# Autodesk Inventor assembly: IMX291 Camera Case Assembly
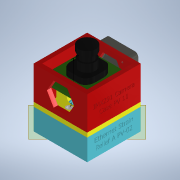
[picture p0: Inventor's stored thumbnail of the model, 180x180]
Saved by Autodesk Inventor 2022.1 (Build 261234000, 234)
## iProperties
Created: 2021-07-23
Part Number: IMX291 Camera Case Assembly
Document SubType Name: Assembly
Designer: robst
Author: robst
## Documents named in this file (10)
- C:\git\CAD-Development\robSteele\ShapeWays\GlobalMeteorNetwork\IMX291 Camera Case Assembly.iam
- C:\git\CAD-Development\robSteele\ShapeWays\GlobalMeteorNetwork\IMX291 Camera Case Base.ipt
- C:\git\CAD-Development\robSteele\ShapeWays\GlobalMeteorNetwork\IMX291 Camera.ipt
- C:\Users\robst\Documents\Inventor\Content Center Files\R2021\en-US\U UNC 2605\Unbrako - 2 x 1_2 - 56(10).ipt
- C:\git\CAD-Development\robSteele\ShapeWays\GlobalMeteorNetwork\IMX291 Camera Case Bottom.ipt
- C:\git\CAD-Development\robSteele\ShapeWays\GlobalMeteorNetwork\IMX291 Ethernet Cable Strain Relief.ipt
- c:\git\CAD-MfgResources\McMaster-Carr\Insert\6-32x0.281_94459A290_NO THREADS_Brass Heat-Set Inserts for Plastic.ipt
- c:\git\CAD-MfgResources\McMaster-Carr\Button Screw\6-32\6-32 x 1_000 92949A153_18-8 Stainless Steel Button Head Hex Drive Screw.ipt
- c:\git\CAD-MfgResources\McMaster-Carr\Washer\Number_6_Washer\90107A007_TYPE 316 STAINLESS STEEL FLAT WASHER.ipt
- C:\git\CAD-Development\robSteele\ShapeWays\GlobalMeteorNetwork\LD3007MS FAN.ipt
## Components (12 placed, 9 different names)
1. IMX291 Camera Case Base:1 — Insert:1, Insert:2, Mate:3, Flush:1, Flush:2, Insert:9, Insert:10
2. IMX291 Camera:1 — Insert:1, Insert:2, Mate:1, Mate:2
3. Unbrako UNC Hex Socket Button Cap - Inch 2 x 1/2:1 — Mate:1, Mate:2
4. IMX291 Camera Case Bottom:1 — Mate:3, Flush:1, Flush:2, Mate:4, Flush:3, Flush:4, Insert:3, Insert:4, Insert:5, Insert:6
5. IMX291 Ethernet Cable Strain Relief:1 — Mate:4, Flush:3, Flush:4, Insert:7
6. 6-32x0.281_94459A290_NO THREADS_Brass Heat-Set Inserts for Plastic:1 — Insert:3
7. 6-32x0.281_94459A290_NO THREADS_Brass Heat-Set Inserts for Plastic:2 — Insert:4
8. 6-32x0.281_94459A290_NO THREADS_Brass Heat-Set Inserts for Plastic:3 — Insert:5
9. 6-32x0.281_94459A290_NO THREADS_Brass Heat-Set Inserts for Plastic:4 — Insert:6
10. 6-32 x 1_000 92949A153_18-8 Stainless Steel Button Head Hex Drive Screw:1 — Insert:8
11. 90107A007_TYPE 316 STAINLESS STEEL FLAT WASHER:1 — Insert:7, Insert:8
12. LD3007MS FAN:1 — Insert:9, Insert:10
## Relationships (18: Insert 10, Mate 4, Flush 4)
- Insert:1: IMX291 Camera Case Base:1 ↔ IMX291 Camera:1
- Insert:2: IMX291 Camera Case Base:1 ↔ IMX291 Camera:1
- Mate:1: IMX291 Camera:1 ↔ Unbrako UNC Hex Socket Button Cap - Inch 2 x 1/2:1
- Mate:2: IMX291 Camera:1 ↔ Unbrako UNC Hex Socket Button Cap - Inch 2 x 1/2:1
- Mate:3: IMX291 Camera Case Base:1 ↔ IMX291 Camera Case Bottom:1
- Flush:1: IMX291 Camera Case Base:1 ↔ IMX291 Camera Case Bottom:1
- Flush:2: IMX291 Camera Case Base:1 ↔ IMX291 Camera Case Bottom:1
- Mate:4: IMX291 Camera Case Bottom:1 ↔ IMX291 Ethernet Cable Strain Relief:1
- Flush:3: IMX291 Camera Case Bottom:1 ↔ IMX291 Ethernet Cable Strain Relief:1
- Flush:4: IMX291 Camera Case Bottom:1 ↔ IMX291 Ethernet Cable Strain Relief:1
- Insert:3: IMX291 Camera Case Bottom:1 ↔ 6-32x0.281_94459A290_NO THREADS_Brass Heat-Set Inserts for Plastic:1
- Insert:4: IMX291 Camera Case Bottom:1 ↔ 6-32x0.281_94459A290_NO THREADS_Brass Heat-Set Inserts for Plastic:2
- Insert:5: IMX291 Camera Case Bottom:1 ↔ 6-32x0.281_94459A290_NO THREADS_Brass Heat-Set Inserts for Plastic:3
- Insert:6: IMX291 Camera Case Bottom:1 ↔ 6-32x0.281_94459A290_NO THREADS_Brass Heat-Set Inserts for Plastic:4
- Insert:7: IMX291 Ethernet Cable Strain Relief:1 ↔ 90107A007_TYPE 316 STAINLESS STEEL FLAT WASHER:1
- Insert:8: 6-32 x 1_000 92949A153_18-8 Stainless Steel Button Head Hex Drive Screw:1 ↔ 90107A007_TYPE 316 STAINLESS STEEL FLAT WASHER:1
- Insert:9: IMX291 Camera Case Base:1 ↔ LD3007MS FAN:1
- Insert:10: IMX291 Camera Case Base:1 ↔ LD3007MS FAN:1
